# Autodesk Inventor assembly: ASY MSC 204 BELLY
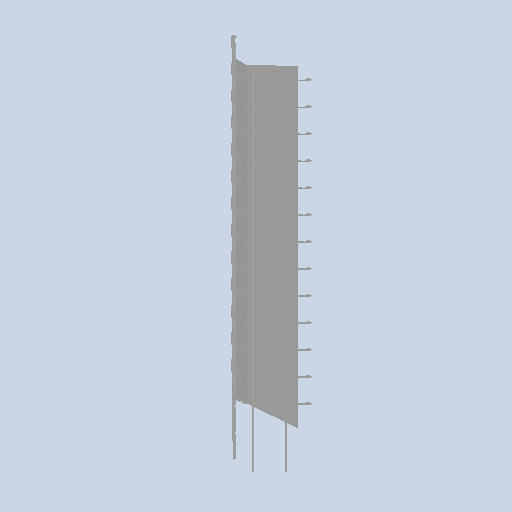
[picture p0: Inventor's stored thumbnail of the model, 512x512]
Saved by Autodesk Inventor 2025 (Build 290162010, 162A)
## iProperties
Created: 2024-07-22
Part Number: ASY MSC 204 BELLY
Document SubType Name: Assembly
Designer: pokla
Author: pokla
## Documents named in this file (5)
- C:\Users\user\YandexDisk\домашниий пк\Inventor\Manturovo\Manturovo_Se-clar\ASY MSC 204 BELLY.iam
- C:\Users\user\YandexDisk\домашниий пк\Inventor\Manturovo\Manturovo_Se-clar\MSC 041 sheet belly main.ipt
- C:\Users\user\YandexDisk\домашниий пк\Inventor\Manturovo\Manturovo_Se-clar\MSC 042 sheet belly-neck.ipt
- C:\Users\user\YandexDisk\домашниий пк\Inventor\Manturovo\Manturovo_Se-clar\MSC 067 stringer board belly.ipt
- C:\Users\user\YandexDisk\домашниий пк\Inventor\Manturovo\Manturovo_Se-clar\MSC 053 rib belly.ipt
## Components (53 placed, 6 different names)
1. MSC 041 sheet belly main.ipt:1
2. MSC 041 sheet belly main.ipt:2
3. MSC 041 sheet belly main.ipt:3
4. MSC 042 sheet belly-neck.ipt:1
5. MSC 041 sheet belly main.ipt:4
6. MSC 041 sheet belly main.ipt:5
7. MSC 041 sheet belly main.ipt:6 — Flush:1, Mate:2
8. MSC 067 stringer board belly.ipt:4
9. MSC 067 stringer board belly.ipt:3
10. MSC 067 stringer board belly.ipt:1
11. MSC 067 stringer board belly.ipt:2
12. MSC 053 rib belly.ipt:2
13. MSC 053 rib belly.ipt:1 — Rigid:17, Flush:1, Mate:1, Mate:2
14. MSC 053 rib belly.ipt:4
15. MSC 053 rib belly.ipt:3 — Rigid:17, Rigid:31
16. MSC 067 stringer board belly.ipt:5 — Rigid:18
17. MSC 067 stringer board belly.ipt:6 — Rigid:23
18. MSC 067 stringer board belly.ipt:8 — Rigid:29
19. MSC 067 stringer board belly.ipt:7 — Rigid:24
20. МОО 057 стрингер борт 7:11 — Rigid:18, Rigid:19
21. МОО 057 стрингер борт 7:12 — Rigid:19, Rigid:20
22. МОО 057 стрингер борт 7:13 — Rigid:20
23. МОО 057 стрингер борт 7:14 — Rigid:23
24. МОО 057 стрингер борт 7:15
25. МОО 057 стрингер борт 7:16
26. МОО 057 стрингер борт 7:17 — Rigid:24, Rigid:25
27. МОО 057 стрингер борт 7:18 — Rigid:25, Rigid:26
28. МОО 057 стрингер борт 7:19 — Rigid:26
29. МОО 057 стрингер борт 7:20 — Rigid:29
30. МОО 057 стрингер борт 7:21
31. МОО 057 стрингер борт 7:22
32. МОО 042 шпангоут брюхо:6
33. МОО 042 шпангоут брюхо:7 — Rigid:31, Rigid:33
34. МОО 042 шпангоут брюхо:8
35. МОО 042 шпангоут брюхо:9 — Rigid:33, Rigid:35
36. МОО 042 шпангоут брюхо:10
37. МОО 042 шпангоут брюхо:11 — Rigid:35, Rigid:41
38. МОО 042 шпангоут брюхо:12
39. МОО 042 шпангоут брюхо:13 — Rigid:41
40. МОО 042 шпангоут брюхо:14
41. МОО 042 шпангоут брюхо:15
42. МОО 042 шпангоут брюхо:16
43. МОО 042 шпангоут брюхо:17 — Rigid:51
44. МОО 042 шпангоут брюхо:18
45. МОО 042 шпангоут брюхо:19 — Rigid:51
46. МОО 042 шпангоут брюхо:20
47. МОО 042 шпангоут брюхо:21
48. МОО 042 шпангоут брюхо:22
49. МОО 042 шпангоут брюхо:23
50. МОО 042 шпангоут брюхо:24
51. МОО 042 шпангоут брюхо:25
52. МОО 042 шпангоут брюхо:26
53. МОО 042 шпангоут брюхо:27
## Relationships (54: WeldJoint 51, Mate 2, Flush 1)
- [WeldJoint]: MSC 041 sheet belly main.ipt:1 ↔ MSC 041 sheet belly main.ipt:2
- [WeldJoint]: MSC 041 sheet belly main.ipt:1 ↔ MSC 041 sheet belly main.ipt:3
- [WeldJoint]: MSC 041 sheet belly main.ipt:4 ↔ MSC 041 sheet belly main.ipt:5
- [WeldJoint]: MSC 041 sheet belly main.ipt:3 ↔ MSC 041 sheet belly main.ipt:4
- [WeldJoint]: MSC 042 sheet belly-neck.ipt:1 ↔ MSC 041 sheet belly main.ipt:5
- [WeldJoint]: MSC 041 sheet belly main.ipt:2 ↔ MSC 041 sheet belly main.ipt:6
- [WeldJoint] (2 mm): MSC 067 stringer board belly.ipt:3 ↔ MSC 053 rib belly.ipt:2
- [WeldJoint] (2 mm): MSC 067 stringer board belly.ipt:1 ↔ MSC 053 rib belly.ipt:1
- [WeldJoint] (2 mm): MSC 067 stringer board belly.ipt:2 ↔ MSC 053 rib belly.ipt:1
- [WeldJoint] (2 mm): MSC 067 stringer board belly.ipt:4 ↔ MSC 053 rib belly.ipt:2
- [WeldJoint] (-50 mm): MSC 053 rib belly.ipt:2 ↔ MSC 053 rib belly.ipt:1
- [WeldJoint] (-50 mm): MSC 053 rib belly.ipt:4 ↔ MSC 053 rib belly.ipt:3
- [WeldJoint]: MSC 067 stringer board belly.ipt:2 ↔ MSC 067 stringer board belly.ipt:8
- [WeldJoint]: MSC 067 stringer board belly.ipt:1 ↔ MSC 067 stringer board belly.ipt:7
- [WeldJoint]: MSC 067 stringer board belly.ipt:3 ↔ MSC 067 stringer board belly.ipt:6
- [WeldJoint]: MSC 067 stringer board belly.ipt:4 ↔ MSC 067 stringer board belly.ipt:5
- Rigid:17 [WeldJoint] (-500 mm): MSC 053 rib belly.ipt:1 ↔ MSC 053 rib belly.ipt:3
- Flush:1 (248 mm): MSC 041 sheet belly main.ipt:6 ↔ MSC 053 rib belly.ipt:1
- Mate:1: MSC 053 rib belly.ipt:1
- Mate:2: MSC 041 sheet belly main.ipt:6 ↔ MSC 053 rib belly.ipt:1
- Rigid:18 [WeldJoint]: MSC 067 stringer board belly.ipt:5 ↔ МОО 057 стрингер борт 7:11
- Rigid:19 [WeldJoint]: МОО 057 стрингер борт 7:11 ↔ МОО 057 стрингер борт 7:12
- Rigid:20 [WeldJoint]: МОО 057 стрингер борт 7:12 ↔ МОО 057 стрингер борт 7:13
- [WeldJoint]: МОО 057 стрингер борт 7:14 ↔ МОО 057 стрингер борт 7:15
- [WeldJoint]: МОО 057 стрингер борт 7:15 ↔ МОО 057 стрингер борт 7:16
- Rigid:23 [WeldJoint]: MSC 067 stringer board belly.ipt:6 ↔ МОО 057 стрингер борт 7:14
- Rigid:24 [WeldJoint]: MSC 067 stringer board belly.ipt:7 ↔ МОО 057 стрингер борт 7:17
- Rigid:25 [WeldJoint]: МОО 057 стрингер борт 7:17 ↔ МОО 057 стрингер борт 7:18
- Rigid:26 [WeldJoint]: МОО 057 стрингер борт 7:18 ↔ МОО 057 стрингер борт 7:19
- [WeldJoint]: МОО 057 стрингер борт 7:20 ↔ МОО 057 стрингер борт 7:21
- [WeldJoint]: МОО 057 стрингер борт 7:21 ↔ МОО 057 стрингер борт 7:22
- Rigid:29 [WeldJoint]: MSC 067 stringer board belly.ipt:8 ↔ МОО 057 стрингер борт 7:20
- [WeldJoint] (-50 mm): МОО 042 шпангоут брюхо:6 ↔ МОО 042 шпангоут брюхо:7
- Rigid:31 [WeldJoint] (-500 mm): MSC 053 rib belly.ipt:3 ↔ МОО 042 шпангоут брюхо:7
- [WeldJoint] (-50 mm): МОО 042 шпангоут брюхо:8 ↔ МОО 042 шпангоут брюхо:9
- Rigid:33 [WeldJoint] (-500 mm): МОО 042 шпангоут брюхо:7 ↔ МОО 042 шпангоут брюхо:9
- [WeldJoint] (-50 mm): МОО 042 шпангоут брюхо:10 ↔ МОО 042 шпангоут брюхо:11
- Rigid:35 [WeldJoint] (-500 mm): МОО 042 шпангоут брюхо:9 ↔ МОО 042 шпангоут брюхо:11
- [WeldJoint] (-50 mm): МОО 042 шпангоут брюхо:12 ↔ МОО 042 шпангоут брюхо:13
- [WeldJoint] (-50 mm): МОО 042 шпангоут брюхо:14 ↔ МОО 042 шпангоут брюхо:15
- [WeldJoint] (-500 mm): МОО 042 шпангоут брюхо:13 ↔ МОО 042 шпангоут брюхо:15
- [WeldJoint] (-50 mm): МОО 042 шпангоут брюхо:16 ↔ МОО 042 шпангоут брюхо:17
- [WeldJoint] (-500 mm): МОО 042 шпангоут брюхо:15 ↔ МОО 042 шпангоут брюхо:17
- Rigid:41 [WeldJoint] (-500 mm): МОО 042 шпангоут брюхо:11 ↔ МОО 042 шпангоут брюхо:13
- [WeldJoint] (-50 mm): МОО 042 шпангоут брюхо:18 ↔ МОО 042 шпангоут брюхо:19
- [WeldJoint] (-50 mm): МОО 042 шпангоут брюхо:20 ↔ МОО 042 шпангоут брюхо:21
- [WeldJoint] (-500 mm): МОО 042 шпангоут брюхо:19 ↔ МОО 042 шпангоут брюхо:21
- [WeldJoint] (-50 mm): МОО 042 шпангоут брюхо:22 ↔ МОО 042 шпангоут брюхо:23
- [WeldJoint] (-50 mm): МОО 042 шпангоут брюхо:24 ↔ МОО 042 шпангоут брюхо:25
- [WeldJoint] (-500 mm): МОО 042 шпангоут брюхо:23 ↔ МОО 042 шпангоут брюхо:25
- [WeldJoint] (-50 mm): МОО 042 шпангоут брюхо:26 ↔ МОО 042 шпангоут брюхо:27
- [WeldJoint] (-500 mm): МОО 042 шпангоут брюхо:25 ↔ МОО 042 шпангоут брюхо:27
- [WeldJoint] (-500 mm): МОО 042 шпангоут брюхо:21 ↔ МОО 042 шпангоут брюхо:23
- Rigid:51 [WeldJoint] (-500 mm): МОО 042 шпангоут брюхо:17 ↔ МОО 042 шпангоут брюхо:19
## Named parameters: d385_d359 = -50 mm, d23_d21 = 0 mm, d24_d22 = 0 mm, d29_d27 = 0 mm, d30_d28 = 0 mm, d32_d385_d359 = -50 mm, d34_d385_d359 = -50 mm, d36_d385_d359 = -50 mm, d38_d32_d385_d359 = -50 mm, d39_d34_d385_d359 = -50 mm, d40_d35 = -500 mm, d41_d36_d385_d359 = -50 mm, d42_d37 = -500 mm, d44_d34_d385_d359 = -50 mm, d45_d36_d385_d359 = -50 mm, d46_d37 = -500 mm, d47_d38_d32_d385_d359 = -50 mm, d48_d39_d34_d385_d359 = -50 mm, d49_d40_d35 = -500 mm, d50_d41_d36_d385_d359 = -50 mm, d51_d42_d37 = -500 mm, d52_d43 = -500 mm
